# Autodesk Inventor assembly: servo mount assembly
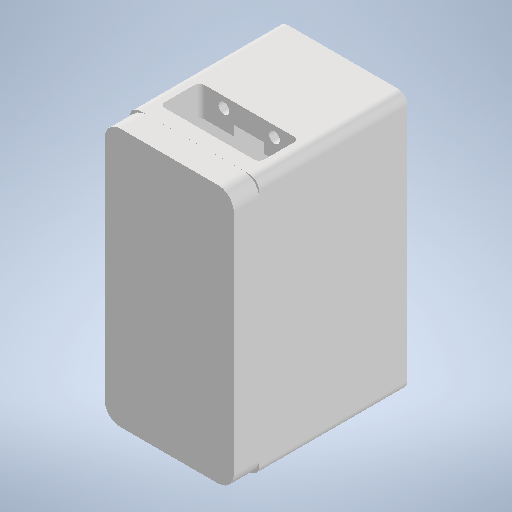
[picture p0: Inventor's stored thumbnail of the model, 512x512]
Saved by Autodesk Inventor 2025.1 (Build 291241000, 241)
## iProperties
Created: 2025-03-10
Part Number: servo mount assembly
Document SubType Name: Assembly
Designer: morai
Author: morai
## Documents named in this file (3)
- C:\Users\morai\Downloads\servo mount assembly.iam
- C:\Users\Public\Documents\Autodesk\Inventor 2025\CAD FILES\FlapFinal v2\4P.01.02.15-BC-v1-Servo Mount.ipt
- C:\Users\Public\Documents\Autodesk\Inventor 2025\CAD FILES\FlapFinal v2\servo mout platform.ipt
## Components (2 placed, 2 different names)
1. 4P.01.02.15-BC-v1-Servo Mount:1 — Rotational:1, Rigid:1
2. servo mout platform:1 — Rotational:1, Rigid:1
## Relationships (2: RevoluteJoint 1, WeldJoint 1)
- Rotational:1 [RevoluteJoint]: 4P.01.02.15-BC-v1-Servo Mount:1 ↔ servo mout platform:1
- Rigid:1 [WeldJoint]: 4P.01.02.15-BC-v1-Servo Mount:1 ↔ servo mout platform:1
